# Autodesk Inventor assembly: CANcoder-Assembled
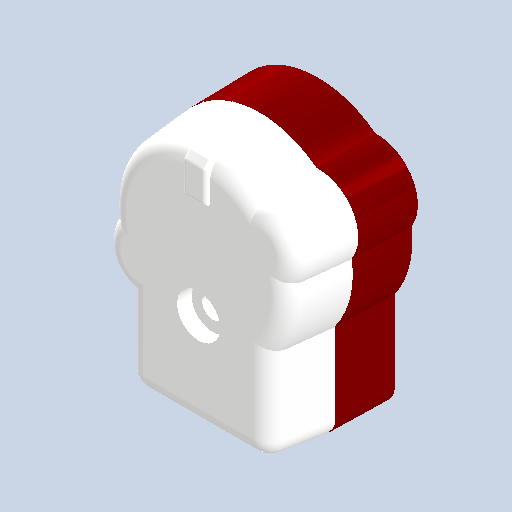
[picture p0: Inventor's stored thumbnail of the model, 512x512]
Saved by Autodesk Inventor 2024 (Build 280153000, 153)
## iProperties
Created: 2024-02-01
Part Number: CANcoder-Assembled
Document SubType Name: Assembly
Designer: rohan
Author: rohan
## Documents named in this file (3)
- C:\Users\5652160\OneDrive - Hillsborough County Public Schools\Robotics\FIRST-Robotics-Competition\Crescendo\Minotaur-Crescendo-Robot\Electronics\CANcoder-Assembled.iam
- C:\Users\5652160\OneDrive - Hillsborough County Public Schools\Robotics\FIRST-Robotics-Competition\Crescendo\Minotaur-Crescendo-Robot\Electronics\CANcoder.iam
- C:\Users\5652160\OneDrive - Hillsborough County Public Schools\Robotics\FIRST-Robotics-Competition\Crescendo\Minotaur-Crescendo-Robot\Structure\3D-Printed-Components\CANcoder-Housing.iam
## Components (2 placed, 2 different names)
1. CANcoder:1 [sub-assembly] — Mate:1, Mate:2
2. CANcoder-Housing:1 [sub-assembly] — Mate:1, Mate:2
## Relationships (2: Mate 2)
- Mate:1: CANcoder:1 ↔ CANcoder-Housing:1
- Mate:2: CANcoder:1 ↔ CANcoder-Housing:1
